# Autodesk Inventor assembly: LinearLift guide custom arm
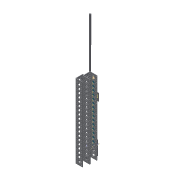
[picture p0: Inventor's stored thumbnail of the model, 180x180]
Saved by Autodesk Inventor 2018 (Build 220112000, 112)
## iProperties
Created: 2017-11-27
Part Number: LinearLift guide custom arm
Document SubType Name: Assembly
Designer: ball
Author: ball
## Documents named in this file (11)
- C:\FTC\FTC8863CAD\2018Robot\LinearLift guide custom arm.iam
- C:\FTC\FTC8863CAD\Actobotics\585 parts\585634.ipt
- C:\FTC\FTC8863CAD\Actobotics\585 parts\585458.ipt
- C:\FTC\FTC8863CAD\2017Robot\LinearBearingPlusClamps.iam
- C:\FTC\FTC8863CAD\Actobotics\634 parts\634315.ipt
- C:\FTC\FTC8863CAD\Actobotics\585 parts\585424.ipt
- C:\FTC\FTC8863CAD\GoBilda\3700 Parts\3700-0145-0288.ipt
- C:\FTC\FTC8863CAD\GoBilda\1609 Parts\1609-0613-0004.ipt
- C:\FTC\FTC8863CAD\GoBilda\2807 Parts\2807-0407-1000.ipt
- C:\FTC\FTC8863CAD\GoBilda\2800 Parts\2800-0004-0016.ipt
- C:\FTC\FTC8863CAD\2018Robot\VWheelArm.ipt
## Components (12 placed, 10 different names)
1. 585458:2 — Mate:44, Angle:1, Mate:49, Mate:50, Mate:51, Mate:54, Mate:55
2. 585634:5 — Mate:44, Flush:5, Mate:47, Mate:48, Mate:54, Mate:55
3. 634315:1 — Flush:5, Mate:46, Mate:48
4. LinearBearingPlusClamps:2 [sub-assembly] — Mate:46, Angle:1, Mate:47, Mate:56, Mate:57, Mate:58
5. 585634:7 — Mate:49, Mate:50, Mate:51
6. 585424:2 — Mate:56, Mate:57, Mate:58, Mate:59, Mate:60, Mate:61, Mate:64
7. 585458:3 — Mate:59, Mate:60, Mate:61, Mate:62, Mate:63
8. 3700-0145-0288:2 — Mate:62, Mate:63, Mate:64, Mate:65, Mate:66
9. 1609-0613-0004:1 — Mate:65, Mate:66, Mate:75, Mate:78, Mate:79, Mate:80
10. 2807-0407-1000:1 — Mate:75, Mate:80, Flush:6
11. 2800-0004-0016:2 — Mate:78, Mate:79
12. VWheelArm:1 — Flush:6
## Relationships (27: Mate 24, Flush 2, Angle 1)
- Mate:44: 585458:2 ↔ 585634:5
- Flush:5: 585634:5 ↔ 634315:1
- Mate:46: 634315:1 ↔ LinearBearingPlusClamps:2
- Angle:1 (0 deg): 585458:2 ↔ LinearBearingPlusClamps:2
- Mate:47: 585634:5 ↔ LinearBearingPlusClamps:2
- Mate:48: 585634:5 ↔ 634315:1
- Mate:49: 585458:2 ↔ 585634:7
- Mate:50: 585458:2 ↔ 585634:7
- Mate:51: 585458:2 ↔ 585634:7
- Mate:54: 585458:2 ↔ 585634:5
- Mate:55: 585458:2 ↔ 585634:5
- Mate:56: LinearBearingPlusClamps:2 ↔ 585424:2
- Mate:57: LinearBearingPlusClamps:2 ↔ 585424:2
- Mate:58: LinearBearingPlusClamps:2 ↔ 585424:2
- Mate:59: 585424:2 ↔ 585458:3
- Mate:60: 585424:2 ↔ 585458:3
- Mate:61: 585424:2 ↔ 585458:3
- Mate:62: 585458:3 ↔ 3700-0145-0288:2
- Mate:63: 585458:3 ↔ 3700-0145-0288:2
- Mate:64: 585424:2 ↔ 3700-0145-0288:2
- Mate:65: 3700-0145-0288:2 ↔ 1609-0613-0004:1
- Mate:66 (11.9888 mm): 3700-0145-0288:2 ↔ 1609-0613-0004:1
- Mate:75: 1609-0613-0004:1 ↔ 2807-0407-1000:1
- Mate:78: 1609-0613-0004:1 ↔ 2800-0004-0016:2
- Mate:79: 1609-0613-0004:1 ↔ 2800-0004-0016:2
- Mate:80: 1609-0613-0004:1 ↔ 2807-0407-1000:1
- Flush:6: 2807-0407-1000:1 ↔ VWheelArm:1
